# Autodesk Inventor assembly: HipUnit
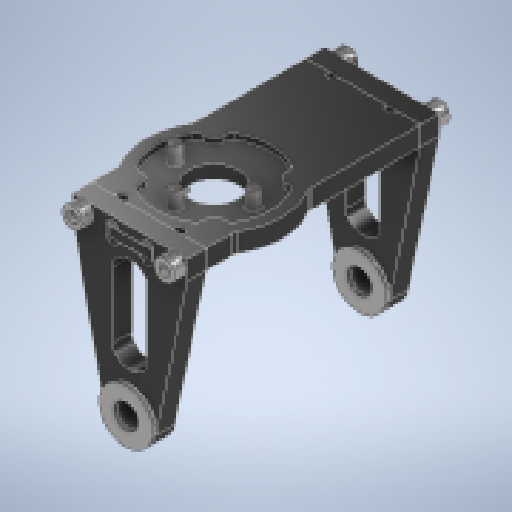
[picture p0: Inventor's stored thumbnail of the model, 512x512]
Saved by Autodesk Inventor 2024.2 (Build 282272000, 272)
## iProperties
Created: 2024-01-04
Part Number: HipUnit
Document SubType Name: Assembly
Designer: Masato Kubotera
Author: Masato Kubotera
## Documents named in this file (7)
- C:\Users\masato\OneDrive - Chiba Institute of Technology\CIT Brains\RoboCup2024\Mechanic\SUSTAINA-OP2\NativeFiles\Boby\LowerLimb\Hips\HipUnit.iam
- C:\Users\masato\OneDrive - Chiba Institute of Technology\CIT Brains\RoboCup2024\Mechanic\SUSTAINA-OP2\NativeFiles\Boby\LowerLimb\LegRollSliderFrame.ipt
- C:\Users\masato\OneDrive - Chiba Institute of Technology\CIT Brains\RoboCup2024\Mechanic\SUSTAINA-OP2\NativeFiles\Boby\LowerLimb\Hips\HipYawJointFrame.ipt
- C:\Users\masato\OneDrive - Chiba Institute of Technology\CIT Brains\RoboCup2024\Mechanic\SUSTAINA-OP2\NativeFiles\Boby\COTS\Screws\CapScrew\UC-0308.ipt
- C:\Users\masato\OneDrive - Chiba Institute of Technology\CIT Brains\RoboCup2024\Mechanic\SUSTAINA-OP2\NativeFiles\Boby\COTS\Bushes\GFM-0608-06.ipt
- C:\Users\masato\OneDrive - Chiba Institute of Technology\CIT Brains\RoboCup2024\Mechanic\SUSTAINA-OP2\NativeFiles\Boby\COTS\Washers\Metal\UUW-0614-05H.ipt
- C:\Users\masato\OneDrive - Chiba Institute of Technology\CIT Brains\RoboCup2024\Mechanic\SUSTAINA-OP2\NativeFiles\Boby\COTS\Washers\Resin\TT-0614-05.ipt
## Components (16 placed, 6 different names)
1. LegRollSliderFrame:1 — Insert:1, Insert:2, Insert:5, Insert:6, Insert:13, Insert:15
2. LegRollSliderFrame:2 — Insert:3, Insert:4, Insert:7, Insert:8, Insert:14, Insert:16
3. HipYawJointFrame:1 — Mate:1, Angle:1, Flush:1, Insert:1, Insert:2, Insert:3, Insert:4, Insert:9, Insert:10, Insert:11
4. UC-0308:1 — Insert:5
5. UC-0308:2 — Insert:6
6. UC-0308:3 — Insert:7
7. UC-0308:4 — Insert:8
8. UC-0308:5 — Insert:9
9. UC-0308:6 — Insert:10
10. UC-0308:7 — Insert:11
11. GFM-0608-06:1 — Insert:13
12. GFM-0608-06:2 — Insert:14
13. TT-0614-05:2 — Insert:15, Insert:17
14. TT-0614-05:1 — Insert:16, Insert:18
15. UUW-0614-05H:1 — Insert:17
16. UUW-0614-05H:2 — Insert:18
## Relationships (20: Insert 17, Mate 1, Angle 1, Flush 1)
- Mate:1: HipYawJointFrame:1
- Angle:1 (0 deg): HipYawJointFrame:1
- Flush:1: HipYawJointFrame:1
- Insert:1: LegRollSliderFrame:1 ↔ HipYawJointFrame:1
- Insert:2: LegRollSliderFrame:1 ↔ HipYawJointFrame:1
- Insert:3: LegRollSliderFrame:2 ↔ HipYawJointFrame:1
- Insert:4: LegRollSliderFrame:2 ↔ HipYawJointFrame:1
- Insert:5: LegRollSliderFrame:1 ↔ UC-0308:1
- Insert:6: LegRollSliderFrame:1 ↔ UC-0308:2
- Insert:7: LegRollSliderFrame:2 ↔ UC-0308:3
- Insert:8: LegRollSliderFrame:2 ↔ UC-0308:4
- Insert:9: HipYawJointFrame:1 ↔ UC-0308:5
- Insert:10: HipYawJointFrame:1 ↔ UC-0308:6
- Insert:11: HipYawJointFrame:1 ↔ UC-0308:7
- Insert:13: LegRollSliderFrame:1 ↔ GFM-0608-06:1
- Insert:14: LegRollSliderFrame:2 ↔ GFM-0608-06:2
- Insert:15: LegRollSliderFrame:1 ↔ TT-0614-05:2
- Insert:16: LegRollSliderFrame:2 ↔ TT-0614-05:1
- Insert:17: TT-0614-05:2 ↔ UUW-0614-05H:1
- Insert:18: TT-0614-05:1 ↔ UUW-0614-05H:2
